# Autodesk Inventor assembly: SplineJoint
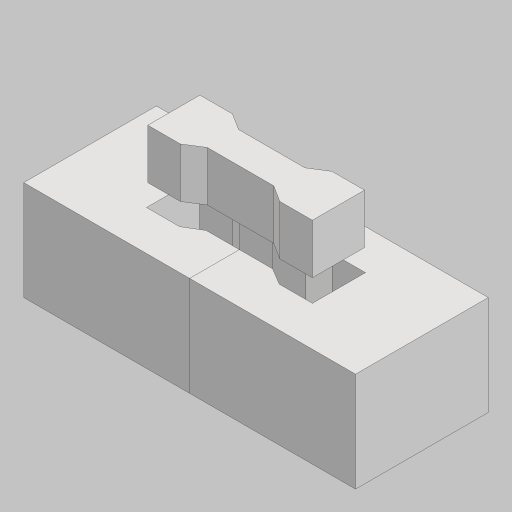
[picture p0: Inventor's stored thumbnail of the model, 512x512]
Saved by Autodesk Inventor 2023 (Build 270158000, 158)
## iProperties
Created: 2026-02-22
Part Number: SplineJoint
Document SubType Name: Assembly
Designer: MARTIN MAESTRE
Author: MARTIN MAESTRE
## Documents named in this file (3)
- C:\Users\MARTIN MAESTRE\OneDrive - Universidad de los Andes\POSTGRADO\202610\MAESTRIA\PROBLEMA ESPECIAL\CADS\Fig3\SplineJoint.iam
- C:\Users\MARTIN MAESTRE\OneDrive - Universidad de los Andes\POSTGRADO\202610\MAESTRIA\PROBLEMA ESPECIAL\CADS\Fig3\Bases.ipt
- C:\Users\MARTIN MAESTRE\OneDrive - Universidad de los Andes\POSTGRADO\202610\MAESTRIA\PROBLEMA ESPECIAL\CADS\Fig3\Spline.ipt
## Components (3 placed, 2 different names)
1. Bases:1 — Coincidencia:1, Coincidencia:2, Coincidencia:3, Coincidencia:4, Nivelación:1, Nivelación:2
2. Bases:2 — Coincidencia:4, Nivelación:1, Nivelación:2, Coincidencia:5, Coincidencia:6
3. Spline:1 — Coincidencia:5, Coincidencia:6
## Relationships (8: Mate 6, Flush 2)
- Coincidencia:1 [Mate]: Bases:1
- Coincidencia:2 [Mate]: Bases:1
- Coincidencia:3 [Mate]: Bases:1
- Coincidencia:4 [Mate]: Bases:1 ↔ Bases:2
- Nivelación:1 [Flush]: Bases:1 ↔ Bases:2
- Nivelación:2 [Flush]: Bases:1 ↔ Bases:2
- Coincidencia:5 [Mate]: Bases:2 ↔ Spline:1
- Coincidencia:6 [Mate]: Bases:2 ↔ Spline:1
